# Autodesk Inventor assembly: PaddleCollection
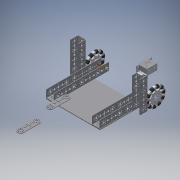
[picture p0: Inventor's stored thumbnail of the model, 180x180]
Saved by Autodesk Inventor 2019 (Build 230136000, 136)
## iProperties
Created: 2018-10-18
Part Number: PaddleCollection
Document SubType Name: Assembly
Designer: User
Author: User
## Documents named in this file (13)
- C:\Robotics\CAD\2018-19_CAD\Collection\PaddleCollection.iam
- C:\Robotics\CAD\COTSParts\Tetrix\Tetrix channel 124 mm.ipt
- C:\Robotics\CAD\COTSParts\Tetrix\Tetrix channel 96mm.ipt
- C:\Robotics\CAD\COTSParts\Tetrix\39274_txm-flat64mmx27mm.ipt
- C:\Robotics\CAD\2018-19_CAD\Collection\PaddleCollectionFloor.ipt
- C:\Robotics\CAD\COTSParts\Tetrix\39060_txm-standard servo bracket.ipt
- C:\Robotics\CAD\COTSParts\Tetrix\Tetrix bracket - angle.ipt
- C:\Robotics\CAD\COTSParts\Tetrix\Tetrix Wheel 3 in omni.ipt
- C:\Robotics\CAD\COTSParts\Tetrix\Bronze bushing.ipt
- C:\Robotics\CAD\COTSParts\Tetrix\Tetrix Hub - axle.ipt
- C:\Robotics\CAD\COTSParts\Tetrix\Tetrix shaft collar.ipt
- C:\Robotics\CAD\COTSParts\Rev\REV-41-1097SmartServo.ipt
- C:\Robotics\CAD\COTSParts\Tetrix\Pitsco Education-739273.ipt
## Components (24 placed, 12 different names)
1. Tetrix channel 124 mm:1 — Insert:3, Flush:6, Insert:9, Insert:11, Insert:19
2. Tetrix channel 124 mm:2 — Insert:1, Flush:5, Flush:7, Insert:5, Insert:8, Insert:10
3. Tetrix channel 96mm:1 — Insert:4, Mate:2, Flush:2, Flush:4, Flush:6
4. Tetrix channel 96mm:2 — Insert:2, Mate:1, Flush:1, Flush:3, Flush:5, Flush:7
5. 39274_txm-flat64mmx27mm:1 — Insert:3, Insert:4
6. 39274_txm-flat64mmx27mm:2 — Insert:1, Insert:2
7. PaddleCollectionFloor:1 — Mate:1, Mate:2, Flush:1, Flush:2, Flush:3, Flush:4, Angle:1, Angle:5
8. Tetrix channel 124 mm:3 — Insert:5, Angle:1, Insert:6, Angle:2
9. 39060_txm-standard servo bracket:1 — Insert:7, Angle:3, Insert:18, Angle:4
10. Tetrix bracket - angle:1 — Insert:6, Angle:2, Insert:7, Angle:3
11. Tetrix Wheel 3 in omni:1 — Insert:17
12. Tetrix Wheel 3 in omni:2 — Insert:15
13. Bronze bushing:1 — Insert:8, Insert:16
14. Bronze bushing:2 — Insert:9, Insert:12
15. Bronze bushing:3 — Insert:11, Insert:14
16. Bronze bushing:4 — Insert:10, Insert:13
17. Tetrix Hub - axle:1 — Insert:16, Insert:17
18. Tetrix Hub - axle:2 — Insert:14, Insert:15
19. Tetrix shaft collar:1 — Insert:13
20. Tetrix shaft collar:2 — Insert:12
21. REV-41-1097SmartServo:1 — Insert:18, Angle:4
22. Tetrix channel 124 mm:4 — Insert:19, Angle:5
23. Pitsco Education-739273:1
24. Pitsco Education-739273:2
## Relationships (33: Insert 19, Flush 7, Angle 5, Mate 2)
- Insert:1: Tetrix channel 124 mm:2 ↔ 39274_txm-flat64mmx27mm:2
- Insert:2: Tetrix channel 96mm:2 ↔ 39274_txm-flat64mmx27mm:2
- Insert:3: Tetrix channel 124 mm:1 ↔ 39274_txm-flat64mmx27mm:1
- Insert:4: Tetrix channel 96mm:1 ↔ 39274_txm-flat64mmx27mm:1
- Mate:1: Tetrix channel 96mm:2 ↔ PaddleCollectionFloor:1
- Mate:2: Tetrix channel 96mm:1 ↔ PaddleCollectionFloor:1
- Flush:1: Tetrix channel 96mm:2 ↔ PaddleCollectionFloor:1
- Flush:2: Tetrix channel 96mm:1 ↔ PaddleCollectionFloor:1
- Flush:3: Tetrix channel 96mm:2 ↔ PaddleCollectionFloor:1
- Flush:4: Tetrix channel 96mm:1 ↔ PaddleCollectionFloor:1
- Flush:5: Tetrix channel 124 mm:2 ↔ Tetrix channel 96mm:2
- Flush:6: Tetrix channel 124 mm:1 ↔ Tetrix channel 96mm:1
- Flush:7: Tetrix channel 124 mm:2 ↔ Tetrix channel 96mm:2
- Insert:5: Tetrix channel 124 mm:2 ↔ Tetrix channel 124 mm:3
- Angle:1 (180 deg): PaddleCollectionFloor:1 ↔ Tetrix channel 124 mm:3
- Insert:6: Tetrix channel 124 mm:3 ↔ Tetrix bracket - angle:1
- Angle:2 (180 deg): Tetrix channel 124 mm:3 ↔ Tetrix bracket - angle:1
- Insert:7: 39060_txm-standard servo bracket:1 ↔ Tetrix bracket - angle:1
- Angle:3 (180 deg): 39060_txm-standard servo bracket:1 ↔ Tetrix bracket - angle:1
- Insert:8: Tetrix channel 124 mm:2 ↔ Bronze bushing:1
- Insert:9: Tetrix channel 124 mm:1 ↔ Bronze bushing:2
- Insert:10: Tetrix channel 124 mm:2 ↔ Bronze bushing:4
- Insert:11: Tetrix channel 124 mm:1 ↔ Bronze bushing:3
- Insert:12: Bronze bushing:2 ↔ Tetrix shaft collar:2
- Insert:13: Bronze bushing:4 ↔ Tetrix shaft collar:1
- Insert:14: Bronze bushing:3 ↔ Tetrix Hub - axle:2
- Insert:15: Tetrix Wheel 3 in omni:2 ↔ Tetrix Hub - axle:2
- Insert:16: Bronze bushing:1 ↔ Tetrix Hub - axle:1
- Insert:17: Tetrix Wheel 3 in omni:1 ↔ Tetrix Hub - axle:1
- Insert:18: 39060_txm-standard servo bracket:1 ↔ REV-41-1097SmartServo:1
- Angle:4 (180 deg): 39060_txm-standard servo bracket:1 ↔ REV-41-1097SmartServo:1
- Insert:19: Tetrix channel 124 mm:1 ↔ Tetrix channel 124 mm:4
- Angle:5 (0 deg): PaddleCollectionFloor:1 ↔ Tetrix channel 124 mm:4
